# Autodesk Inventor assembly: RobotMK2
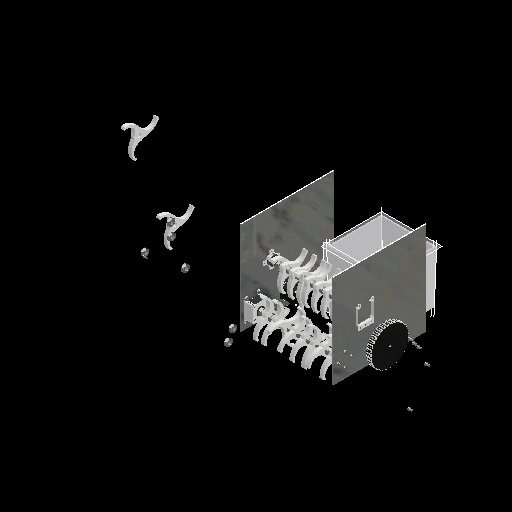
[picture p0: Inventor's stored thumbnail of the model, 512x512]
Saved by Autodesk Inventor 2025 (Build 290162000, 162)
## iProperties
Created: 2025-01-19
Part Number: RobotMK2
Document SubType Name: Assembly
Designer: Trevor
Author: Trevor
## Documents named in this file (18)
- C:\Users\Trevor\Documents\GitHub\USA-Robotic-Club-2024\assests\RobotMK2.iam
- C:\Users\Trevor\Documents\GitHub\USA-Robotic-Club-2024\assests\RightALPanel.ipt
- C:\Users\Trevor\Documents\GitHub\USA-Robotic-Club-2024\assests\LeftALPanel.ipt
- C:\Users\Trevor\Documents\GitHub\USA-Robotic-Club-2024\assests\RobotWheelMK1.ipt
- C:\Users\Trevor\Documents\GitHub\USA-Robotic-Club-2024\assests\Robot Box.ipt
- C:\Users\Trevor\Documents\GitHub\USA-Robotic-Club-2024\assests\17hm08-1204s-nema17-pancake-21mm-1.snapshot.2\17HM08-1204S Nema17 Pancake 21mm\17HM08-1204S Nema17 Pancake 21mm.ipt
- C:\Users\Trevor\Documents\GitHub\USA-Robotic-Club-2024\assests\stepperonline-nema-17-1.snapshot.1\Stepper Motor\Stepper Motor.ipt
- C:\Users\Trevor\Documents\GitHub\USA-Robotic-Club-2024\assests\RodMK3.ipt
- C:\Users\Trevor\Documents\GitHub\USA-Robotic-Club-2024\assests\Combine mk5.ipt
- C:\Users\Trevor\Documents\GitHub\USA-Robotic-Club-2024\assests\bearing-10mm-2.snapshot.2\PMG(Si)\PMG(Si).ipt
- C:\Users\Trevor\Documents\Inventor\Content Center Files\R2025\en-US\DIN 934\DIN 934 - M10 x 1.ipt
- C:\Users\Trevor\Documents\GitHub\USA-Robotic-Club-2024\assests\PanpackeMotorMountMK2.ipt
- C:\Users\Trevor\Documents\GitHub\USA-Robotic-Club-2024\assests\BearingMountMK2.ipt
- C:\Users\Trevor\Documents\Inventor\Content Center Files\R2025\en-US\ANSI B18.3.4M(1)\ANSI B18.3.4M - M5 x 0.8 x 8(2).ipt
- C:\Users\Trevor\Documents\Inventor\Content Center Files\R2025\en-US\DIN 934\DIN 934 - M5 x 0.8.ipt
- C:\Users\Trevor\Documents\Inventor\Content Center Files\R2025\en-US\ANSI B18.3.4M(1)\ANSI B18.3.4M - M3 x 0.5 x 10(2).ipt
- C:\Users\Trevor\Documents\Inventor\Content Center Files\R2025\en-US\ANSI B18.3.4M(1)\ANSI B18.3.4M - M5 x 0.8 x 10(2).ipt
- C:\Users\Trevor\Documents\GitHub\USA-Robotic-Club-2024\assests\Bucket no fillets 2.ipt
## Components (108 placed, 17 different names)
1. Robot Box:1 — Mate:1, Mate:2, Mate:3, Mate:4, Mate:5, Mate:6, Mate:7, Flush:3, Flush:4, Mate:12
2. RobotWheelMK1:1 — Mate:2, Mate:3, Mate:4, Flush:1, Mate:8
3. RobotWheelMK1:2 — Mate:5, Mate:6, Mate:7, Mate:10
4. RightALPanel:1 — Flush:5, Mate:9, Mate:21, Flush:11, Mate:74, Mate:76, Mate:77, Mate:79, Mate:81, Mate:82, Mate:83, Mate:88, Mate:91, Mate:92, Mate:93, Mate:94, Mate:95, Mate:96, Mate:97, Mate:131
5. LeftALPanel:1 — Flush:6, Mate:11, Mate:17, Flush:7, Flush:10, Mate:98, Mate:99, Mate:100, Mate:101, Mate:102, Mate:103, Mate:104, Mate:105, Mate:106, Mate:107, Mate:108, Mate:116, Mate:117, Mate:118, Mate:122, Mate:124, Mate:127, Mate:128, Mate:129, Mate:132, Mate:133
6. Stepper Motor:1 — Mate:8, Mate:9, Mate:13, Mate:90
7. Stepper Motor:2 — Mate:10, Mate:11, Mate:12, Mate:13
8. RodMK3:1 — Mate:18, Mate:19, Mate:20, Mate:24, Mate:26, Mate:28, Mate:29, Mate:30, Mate:31, Mate:33, Mate:34, Mate:38, Mate:39, Mate:43, Mate:44, Mate:48, Mate:50, Mate:52, Mate:54, Mate:55, Mate:58, Mate:60, Mate:61, Mate:64, Mate:66, Mate:67, Mate:70, Mate:72
9. 17HM08-1204S Nema17 Pancake 21mm:1 — Mate:17, Mate:18, Mate:19, Flush:8, Flush:9
10. PMG(Si):1 — Mate:20, Mate:21
11. DIN 934 - replaced by DIN EN 24032/28673/28674 M10 x 1:1 — Mate:24, Mate:27
12. DIN 934 - replaced by DIN EN 24032/28673/28674 M10 x 1:2 — Mate:26, Mate:27, Mate:32
13. DIN 934 - replaced by DIN EN 24032/28673/28674 M10 x 1:4 — Mate:48, Mate:49, Mate:51
14. DIN 934 - replaced by DIN EN 24032/28673/28674 M10 x 1:3 — Mate:33, Mate:35, Mate:36
15. DIN 934 - replaced by DIN EN 24032/28673/28674 M10 x 1:5 — Mate:34, Mate:36, Mate:37
16. DIN 934 - replaced by DIN EN 24032/28673/28674 M10 x 1:6 — Mate:38, Mate:40, Mate:41
17. DIN 934 - replaced by DIN EN 24032/28673/28674 M10 x 1:7 — Mate:50, Mate:51, Mate:53
18. DIN 934 - replaced by DIN EN 24032/28673/28674 M10 x 1:8 — Mate:44, Mate:46, Mate:47
19. DIN 934 - replaced by DIN EN 24032/28673/28674 M10 x 1:9 — Mate:43, Mate:45, Mate:46
20. DIN 934 - replaced by DIN EN 24032/28673/28674 M10 x 1:10 — Mate:39, Mate:41, Mate:42
21. DIN 934 - replaced by DIN EN 24032/28673/28674 M10 x 1:11 — Mate:60, Mate:62, Mate:63
22. DIN 934 - replaced by DIN EN 24032/28673/28674 M10 x 1:12 — Mate:66, Mate:68, Mate:69
23. Combine mk5:2 — Mate:28, Mate:32, Mate:35
24. Combine mk5:3 — Mate:29, Mate:37, Mate:40
25. Combine mk5:4 — Mate:30, Mate:42, Mate:45
26. Combine mk5:5 — Mate:31, Mate:47, Mate:49
27. Combine mk5:6 — Mate:146, Mate:147, Mate:149
28. Combine mk5:7 — Mate:70, Mate:71, Mate:73
29. Combine mk5:8 — Mate:58, Mate:59, Mate:62
30. Combine mk5:9 — Mate:64, Mate:65, Mate:68
31. Combine mk5:10 — Mate:140, Mate:141, Mate:143
32. Combine mk5:11 — Mate:52, Mate:53, Mate:56
33. DIN 934 - replaced by DIN EN 24032/28673/28674 M10 x 1:13 — Mate:61, Mate:63, Mate:65
34. DIN 934 - replaced by DIN EN 24032/28673/28674 M10 x 1:14 — Mate:67, Mate:69, Mate:71
35. DIN 934 - replaced by DIN EN 24032/28673/28674 M10 x 1:15 — Mate:160, Mate:161, Mate:163
36. DIN 934 - replaced by DIN EN 24032/28673/28674 M10 x 1:16 — Mate:144, Mate:145, Mate:147
37. DIN 934 - replaced by DIN EN 24032/28673/28674 M10 x 1:17 — Mate:54, Mate:56, Mate:57
38. DIN 934 - replaced by DIN EN 24032/28673/28674 M10 x 1:18 — Mate:55, Mate:57, Mate:59
39. DIN 934 - replaced by DIN EN 24032/28673/28674 M10 x 1:19 — Mate:72, Mate:73
40. DIN 934 - replaced by DIN EN 24032/28673/28674 M10 x 1:20 — Mate:138, Mate:139, Mate:141
41. DIN 934 - replaced by DIN EN 24032/28673/28674 M10 x 1:21 — Mate:142, Mate:143, Mate:145
42. PanpackeMotorMountMK2:1 — Flush:9, Flush:10, Mate:109, Mate:110, Mate:111, Mate:112, Mate:113, Mate:114, Mate:115
43. BearingMountMK2:1 — Flush:11, Mate:75, Mate:78, Mate:80, Mate:126
44. Broached Hexagon Socket Button Head Cap Screw - Metric M5 x 0.8 x 10:8 — Mate:74, Mate:75, Mate:84
45. Broached Hexagon Socket Button Head Cap Screw - Metric M5 x 0.8 x 10:9 — Mate:76, Mate:85, Mate:126
46. Broached Hexagon Socket Button Head Cap Screw - Metric M5 x 0.8 x 8:3
47. Broached Hexagon Socket Button Head Cap Screw - Metric M5 x 0.8 x 10:1 — Mate:106, Mate:115, Mate:125
48. Broached Hexagon Socket Button Head Cap Screw - Metric M5 x 0.8 x 10:7 — Mate:77, Mate:78, Mate:89
49. Broached Hexagon Socket Button Head Cap Screw - Metric M5 x 0.8 x 8:6
50. Broached Hexagon Socket Button Head Cap Screw - Metric M5 x 0.8 x 8:7
51. Broached Hexagon Socket Button Head Cap Screw - Metric M5 x 0.8 x 10:6 — Mate:79, Mate:80, Mate:87
52. Broached Hexagon Socket Button Head Cap Screw - Metric M5 x 0.8 x 8:9
53. Broached Hexagon Socket Button Head Cap Screw - Metric M5 x 0.8 x 8:10
54. DIN 934 - replaced by DIN EN 24032/28673/28674 M5:1 — Mate:82, Mate:85
55. DIN 934 - replaced by DIN EN 24032/28673/28674 M5:2 — Mate:81, Mate:84
56. DIN 934 - replaced by DIN EN 24032/28673/28674 M5:4 — Mate:83, Mate:87
57. DIN 934 - replaced by DIN EN 24032/28673/28674 M5:5 — Mate:88, Mate:89
58. Broached Hexagon Socket Button Head Cap Screw - Metric M3 x 0.5 x 10:1 — Mate:94, Mate:96
59. Broached Hexagon Socket Button Head Cap Screw - Metric M3 x 0.5 x 10:2 — Mate:93, Mate:95
60. Broached Hexagon Socket Button Head Cap Screw - Metric M3 x 0.5 x 10:3
61. Broached Hexagon Socket Button Head Cap Screw - Metric M3 x 0.5 x 10:4 — Mate:92, Mate:97
62. Broached Hexagon Socket Button Head Cap Screw - Metric M3 x 0.5 x 10:5 — Mate:90, Mate:91
63. Broached Hexagon Socket Button Head Cap Screw - Metric M3 x 0.5 x 10:7 — Mate:98, Mate:102
64. Broached Hexagon Socket Button Head Cap Screw - Metric M3 x 0.5 x 10:8 — Mate:99, Mate:104
65. Broached Hexagon Socket Button Head Cap Screw - Metric M3 x 0.5 x 10:9 — Mate:100, Mate:105
66. Broached Hexagon Socket Button Head Cap Screw - Metric M3 x 0.5 x 10:10 — Mate:101, Mate:103
67. Broached Hexagon Socket Button Head Cap Screw - Metric M5 x 0.8 x 10:2 — Mate:107, Mate:114, Mate:121
68. Broached Hexagon Socket Button Head Cap Screw - Metric M5 x 0.8 x 10:3 — Mate:108, Mate:113, Mate:123
69. Broached Hexagon Socket Button Head Cap Screw - Metric M5 x 0.8 x 10:4 — Mate:109, Mate:112, Mate:119
70. Broached Hexagon Socket Button Head Cap Screw - Metric M5 x 0.8 x 10:5 — Mate:110, Mate:111, Mate:120
71. DIN 934 - replaced by DIN EN 24032/28673/28674 M5:6 — Mate:118, Mate:121
72. DIN 934 - replaced by DIN EN 24032/28673/28674 M5:7 — Mate:117, Mate:119
73. DIN 934 - replaced by DIN EN 24032/28673/28674 M5:8 — Mate:122, Mate:123
74. DIN 934 - replaced by DIN EN 24032/28673/28674 M5:10 — Mate:116, Mate:120
75. DIN 934 - replaced by DIN EN 24032/28673/28674 M5:11 — Mate:124, Mate:125
76. PanpackeMotorMountMK2:2 — Mate:136, Mate:137
77. PMG(Si):2 — Mate:127, Mate:128, Mate:130
78. BearingMountMK2:2 — Mate:129, Mate:130
79. RodMK3:2 — Mate:133, Mate:134, Mate:135, Mate:138, Mate:140, Mate:142, Mate:144, Mate:146, Mate:148, Mate:150, Mate:152, Mate:154, Mate:155, Mate:157, Mate:160, Mate:162, Mate:164, Mate:166, Mate:168, Mate:170, Mate:171, Mate:172, Mate:175, Mate:177, Mate:178, Mate:181, Mate:183, Mate:184
80. 17HM08-1204S Nema17 Pancake 21mm:2 — Mate:131, Mate:132, Mate:134, Mate:135, Mate:136, Mate:137, Mate:139
81. DIN 934 - replaced by DIN EN 24032/28673/28674 M10 x 1:22 — Mate:148, Mate:149, Mate:151
82. DIN 934 - replaced by DIN EN 24032/28673/28674 M10 x 1:23 — Mate:150, Mate:151, Mate:153
83. DIN 934 - replaced by DIN EN 24032/28673/28674 M10 x 1:24 — Mate:155, Mate:156, Mate:158
84. DIN 934 - replaced by DIN EN 24032/28673/28674 M10 x 1:25 — Mate:157, Mate:158, Mate:159
85. DIN 934 - replaced by DIN EN 24032/28673/28674 M10 x 1:26 — Mate:162, Mate:163, Mate:165
86. DIN 934 - replaced by DIN EN 24032/28673/28674 M10 x 1:27
87. Combine mk5:12 — Mate:152, Mate:153, Mate:156
88. Combine mk5:13 — Mate:154, Mate:159, Mate:161
89. Combine mk5:14 — Mate:164, Mate:165, Mate:167
90. Combine mk5:15 — Mate:170, Mate:173
91. Combine mk5:16
92. Combine mk5:17 — Mate:181, Mate:182, Mate:185
93. Combine mk5:19 — Mate:175, Mate:176, Mate:179
94. Combine mk5:20
95. DIN 934 - replaced by DIN EN 24032/28673/28674 M10 x 1:28
96. DIN 934 - replaced by DIN EN 24032/28673/28674 M10 x 1:29 — Mate:168, Mate:169
97. DIN 934 - replaced by DIN EN 24032/28673/28674 M10 x 1:30 — Mate:178, Mate:179, Mate:180
98. DIN 934 - replaced by DIN EN 24032/28673/28674 M10 x 1:31 — Mate:172, Mate:174, Mate:176
99. DIN 934 - replaced by DIN EN 24032/28673/28674 M10 x 1:32
100. DIN 934 - replaced by DIN EN 24032/28673/28674 M10 x 1:33 — Mate:184, Mate:186
101. DIN 934 - replaced by DIN EN 24032/28673/28674 M10 x 1:34
102. DIN 934 - replaced by DIN EN 24032/28673/28674 M10 x 1:36 — Mate:171, Mate:173, Mate:174
103. DIN 934 - replaced by DIN EN 24032/28673/28674 M10 x 1:37 — Mate:183, Mate:185, Mate:186
104. DIN 934 - replaced by DIN EN 24032/28673/28674 M10 x 1:38 — Mate:166, Mate:167, Mate:169
105. DIN 934 - replaced by DIN EN 24032/28673/28674 M10 x 1:39
106. DIN 934 - replaced by DIN EN 24032/28673/28674 M10 x 1:40
107. DIN 934 - replaced by DIN EN 24032/28673/28674 M10 x 1:41 — Mate:177, Mate:180, Mate:182
108. Bucket no fillets 2:1
## Relationships (189: Mate 179, Flush 10)
- Mate:1: Robot Box:1
- Mate:2: Robot Box:1 ↔ RobotWheelMK1:1
- Mate:3 (2 mm): Robot Box:1 ↔ RobotWheelMK1:1
- Mate:4: Robot Box:1 ↔ RobotWheelMK1:1
- Mate:5: Robot Box:1 ↔ RobotWheelMK1:2
- Mate:6 (2 mm): Robot Box:1 ↔ RobotWheelMK1:2
- Mate:7: Robot Box:1 ↔ RobotWheelMK1:2
- Flush:1 (2 mm): RobotWheelMK1:1
- Flush:3 (20 mm): Robot Box:1
- Flush:4 (30 mm): Robot Box:1
- Flush:5: RightALPanel:1
- Flush:6: LeftALPanel:1
- Mate:8: RobotWheelMK1:1 ↔ Stepper Motor:1
- Mate:9: RightALPanel:1 ↔ Stepper Motor:1
- Mate:10: RobotWheelMK1:2 ↔ Stepper Motor:2
- Mate:11: LeftALPanel:1 ↔ Stepper Motor:2
- Mate:12: Robot Box:1 ↔ Stepper Motor:2
- Mate:13: Stepper Motor:1 ↔ Stepper Motor:2
- Mate:17: LeftALPanel:1 ↔ 17HM08-1204S Nema17 Pancake 21mm:1
- Mate:18: RodMK3:1 ↔ 17HM08-1204S Nema17 Pancake 21mm:1
- Mate:19: RodMK3:1 ↔ 17HM08-1204S Nema17 Pancake 21mm:1
- Flush:7 (-10 mm): LeftALPanel:1
- Flush:8: 17HM08-1204S Nema17 Pancake 21mm:1
- Mate:20: RodMK3:1 ↔ PMG(Si):1
- Mate:21: RightALPanel:1 ↔ PMG(Si):1
- Mate:24: RodMK3:1 ↔ DIN 934 - replaced by DIN EN 24032/28673/28674 M10 x 1:1
- Mate:26: RodMK3:1 ↔ DIN 934 - replaced by DIN EN 24032/28673/28674 M10 x 1:2
- Mate:27: DIN 934 - replaced by DIN EN 24032/28673/28674 M10 x 1:1 ↔ DIN 934 - replaced by DIN EN 24032/28673/28674 M10 x 1:2
- Mate:28: RodMK3:1 ↔ Combine mk5:2
- Mate:29: RodMK3:1 ↔ Combine mk5:3
- Mate:30: RodMK3:1 ↔ Combine mk5:4
- Mate:31: RodMK3:1 ↔ Combine mk5:5
- Mate:32: DIN 934 - replaced by DIN EN 24032/28673/28674 M10 x 1:2 ↔ Combine mk5:2
- Mate:33: RodMK3:1 ↔ DIN 934 - replaced by DIN EN 24032/28673/28674 M10 x 1:3
- Mate:34: RodMK3:1 ↔ DIN 934 - replaced by DIN EN 24032/28673/28674 M10 x 1:5
- Mate:35: DIN 934 - replaced by DIN EN 24032/28673/28674 M10 x 1:3 ↔ Combine mk5:2
- Mate:36: DIN 934 - replaced by DIN EN 24032/28673/28674 M10 x 1:3 ↔ DIN 934 - replaced by DIN EN 24032/28673/28674 M10 x 1:5
- Mate:37: DIN 934 - replaced by DIN EN 24032/28673/28674 M10 x 1:5 ↔ Combine mk5:3
- Mate:38: RodMK3:1 ↔ DIN 934 - replaced by DIN EN 24032/28673/28674 M10 x 1:6
- Mate:39: RodMK3:1 ↔ DIN 934 - replaced by DIN EN 24032/28673/28674 M10 x 1:10
- Mate:40: DIN 934 - replaced by DIN EN 24032/28673/28674 M10 x 1:6 ↔ Combine mk5:3
- Mate:41: DIN 934 - replaced by DIN EN 24032/28673/28674 M10 x 1:6 ↔ DIN 934 - replaced by DIN EN 24032/28673/28674 M10 x 1:10
- Mate:42: DIN 934 - replaced by DIN EN 24032/28673/28674 M10 x 1:10 ↔ Combine mk5:4
- Mate:43: RodMK3:1 ↔ DIN 934 - replaced by DIN EN 24032/28673/28674 M10 x 1:9
- Mate:44: RodMK3:1 ↔ DIN 934 - replaced by DIN EN 24032/28673/28674 M10 x 1:8
- Mate:45: DIN 934 - replaced by DIN EN 24032/28673/28674 M10 x 1:9 ↔ Combine mk5:4
- Mate:46: DIN 934 - replaced by DIN EN 24032/28673/28674 M10 x 1:8 ↔ DIN 934 - replaced by DIN EN 24032/28673/28674 M10 x 1:9
- Mate:47: DIN 934 - replaced by DIN EN 24032/28673/28674 M10 x 1:8 ↔ Combine mk5:5
- Mate:48: RodMK3:1 ↔ DIN 934 - replaced by DIN EN 24032/28673/28674 M10 x 1:4
- Mate:49: DIN 934 - replaced by DIN EN 24032/28673/28674 M10 x 1:4 ↔ Combine mk5:5
- Mate:50: RodMK3:1 ↔ DIN 934 - replaced by DIN EN 24032/28673/28674 M10 x 1:7
- Mate:51: DIN 934 - replaced by DIN EN 24032/28673/28674 M10 x 1:4 ↔ DIN 934 - replaced by DIN EN 24032/28673/28674 M10 x 1:7
- Mate:52: RodMK3:1 ↔ Combine mk5:11
- Mate:53: DIN 934 - replaced by DIN EN 24032/28673/28674 M10 x 1:7 ↔ Combine mk5:11
- Mate:54: RodMK3:1 ↔ DIN 934 - replaced by DIN EN 24032/28673/28674 M10 x 1:17
- Mate:55: RodMK3:1 ↔ DIN 934 - replaced by DIN EN 24032/28673/28674 M10 x 1:18
- Mate:56: Combine mk5:11 ↔ DIN 934 - replaced by DIN EN 24032/28673/28674 M10 x 1:17
- Mate:57: DIN 934 - replaced by DIN EN 24032/28673/28674 M10 x 1:17 ↔ DIN 934 - replaced by DIN EN 24032/28673/28674 M10 x 1:18
- Mate:58: RodMK3:1 ↔ Combine mk5:8
- Mate:59: Combine mk5:8 ↔ DIN 934 - replaced by DIN EN 24032/28673/28674 M10 x 1:18
- Mate:60: RodMK3:1 ↔ DIN 934 - replaced by DIN EN 24032/28673/28674 M10 x 1:11
- Mate:61: RodMK3:1 ↔ DIN 934 - replaced by DIN EN 24032/28673/28674 M10 x 1:13
- Mate:62: DIN 934 - replaced by DIN EN 24032/28673/28674 M10 x 1:11 ↔ Combine mk5:8
- Mate:63: DIN 934 - replaced by DIN EN 24032/28673/28674 M10 x 1:11 ↔ DIN 934 - replaced by DIN EN 24032/28673/28674 M10 x 1:13
- Mate:64: RodMK3:1 ↔ Combine mk5:9
- Mate:65: Combine mk5:9 ↔ DIN 934 - replaced by DIN EN 24032/28673/28674 M10 x 1:13
- Mate:66: RodMK3:1 ↔ DIN 934 - replaced by DIN EN 24032/28673/28674 M10 x 1:12
- Mate:67: RodMK3:1 ↔ DIN 934 - replaced by DIN EN 24032/28673/28674 M10 x 1:14
- Mate:68: DIN 934 - replaced by DIN EN 24032/28673/28674 M10 x 1:12 ↔ Combine mk5:9
- Mate:69: DIN 934 - replaced by DIN EN 24032/28673/28674 M10 x 1:12 ↔ DIN 934 - replaced by DIN EN 24032/28673/28674 M10 x 1:14
- Mate:70: RodMK3:1 ↔ Combine mk5:7
- Mate:71: Combine mk5:7 ↔ DIN 934 - replaced by DIN EN 24032/28673/28674 M10 x 1:14
- Mate:72: RodMK3:1 ↔ DIN 934 - replaced by DIN EN 24032/28673/28674 M10 x 1:19
- Mate:73: Combine mk5:7 ↔ DIN 934 - replaced by DIN EN 24032/28673/28674 M10 x 1:19
- Flush:9: 17HM08-1204S Nema17 Pancake 21mm:1 ↔ PanpackeMotorMountMK2:1
- Flush:10: LeftALPanel:1 ↔ PanpackeMotorMountMK2:1
- Flush:11: RightALPanel:1 ↔ BearingMountMK2:1
- Mate:74: RightALPanel:1 ↔ Broached Hexagon Socket Button Head Cap Screw - Metric M5 x 0.8 x 10:8
- Mate:75: BearingMountMK2:1 ↔ Broached Hexagon Socket Button Head Cap Screw - Metric M5 x 0.8 x 10:8
- Mate:76: RightALPanel:1 ↔ Broached Hexagon Socket Button Head Cap Screw - Metric M5 x 0.8 x 10:9
- Mate:77: RightALPanel:1 ↔ Broached Hexagon Socket Button Head Cap Screw - Metric M5 x 0.8 x 10:7
- Mate:78: BearingMountMK2:1 ↔ Broached Hexagon Socket Button Head Cap Screw - Metric M5 x 0.8 x 10:7
- Mate:79: RightALPanel:1 ↔ Broached Hexagon Socket Button Head Cap Screw - Metric M5 x 0.8 x 10:6
- Mate:80: BearingMountMK2:1 ↔ Broached Hexagon Socket Button Head Cap Screw - Metric M5 x 0.8 x 10:6
- Mate:81: RightALPanel:1 ↔ DIN 934 - replaced by DIN EN 24032/28673/28674 M5:2
- Mate:82: RightALPanel:1 ↔ DIN 934 - replaced by DIN EN 24032/28673/28674 M5:1
- Mate:83: RightALPanel:1 ↔ DIN 934 - replaced by DIN EN 24032/28673/28674 M5:4
- Mate:84: Broached Hexagon Socket Button Head Cap Screw - Metric M5 x 0.8 x 10:8 ↔ DIN 934 - replaced by DIN EN 24032/28673/28674 M5:2
- Mate:85: Broached Hexagon Socket Button Head Cap Screw - Metric M5 x 0.8 x 10:9 ↔ DIN 934 - replaced by DIN EN 24032/28673/28674 M5:1
- Mate:87: Broached Hexagon Socket Button Head Cap Screw - Metric M5 x 0.8 x 10:6 ↔ DIN 934 - replaced by DIN EN 24032/28673/28674 M5:4
- Mate:88: RightALPanel:1 ↔ DIN 934 - replaced by DIN EN 24032/28673/28674 M5:5
- Mate:89: Broached Hexagon Socket Button Head Cap Screw - Metric M5 x 0.8 x 10:7 ↔ DIN 934 - replaced by DIN EN 24032/28673/28674 M5:5
- Mate:90: Stepper Motor:1 ↔ Broached Hexagon Socket Button Head Cap Screw - Metric M3 x 0.5 x 10:5
- Mate:91: RightALPanel:1 ↔ Broached Hexagon Socket Button Head Cap Screw - Metric M3 x 0.5 x 10:5
- Mate:92: RightALPanel:1 ↔ Broached Hexagon Socket Button Head Cap Screw - Metric M3 x 0.5 x 10:4
- Mate:93: RightALPanel:1 ↔ Broached Hexagon Socket Button Head Cap Screw - Metric M3 x 0.5 x 10:2
- Mate:94: RightALPanel:1 ↔ Broached Hexagon Socket Button Head Cap Screw - Metric M3 x 0.5 x 10:1
- Mate:95: RightALPanel:1 ↔ Broached Hexagon Socket Button Head Cap Screw - Metric M3 x 0.5 x 10:2
- Mate:96: RightALPanel:1 ↔ Broached Hexagon Socket Button Head Cap Screw - Metric M3 x 0.5 x 10:1
- Mate:97: RightALPanel:1 ↔ Broached Hexagon Socket Button Head Cap Screw - Metric M3 x 0.5 x 10:4
- Mate:98: LeftALPanel:1 ↔ Broached Hexagon Socket Button Head Cap Screw - Metric M3 x 0.5 x 10:7
- Mate:99: LeftALPanel:1 ↔ Broached Hexagon Socket Button Head Cap Screw - Metric M3 x 0.5 x 10:8
- Mate:100: LeftALPanel:1 ↔ Broached Hexagon Socket Button Head Cap Screw - Metric M3 x 0.5 x 10:9
- Mate:101: LeftALPanel:1 ↔ Broached Hexagon Socket Button Head Cap Screw - Metric M3 x 0.5 x 10:10
- Mate:102: LeftALPanel:1 ↔ Broached Hexagon Socket Button Head Cap Screw - Metric M3 x 0.5 x 10:7
- Mate:103: LeftALPanel:1 ↔ Broached Hexagon Socket Button Head Cap Screw - Metric M3 x 0.5 x 10:10
- Mate:104: LeftALPanel:1 ↔ Broached Hexagon Socket Button Head Cap Screw - Metric M3 x 0.5 x 10:8
- Mate:105: LeftALPanel:1 ↔ Broached Hexagon Socket Button Head Cap Screw - Metric M3 x 0.5 x 10:9
- Mate:106: LeftALPanel:1 ↔ Broached Hexagon Socket Button Head Cap Screw - Metric M5 x 0.8 x 10:1
- Mate:107: LeftALPanel:1 ↔ Broached Hexagon Socket Button Head Cap Screw - Metric M5 x 0.8 x 10:2
- Mate:108: LeftALPanel:1 ↔ Broached Hexagon Socket Button Head Cap Screw - Metric M5 x 0.8 x 10:3
- Mate:109: PanpackeMotorMountMK2:1 ↔ Broached Hexagon Socket Button Head Cap Screw - Metric M5 x 0.8 x 10:4
- Mate:110: PanpackeMotorMountMK2:1 ↔ Broached Hexagon Socket Button Head Cap Screw - Metric M5 x 0.8 x 10:5
- Mate:111: PanpackeMotorMountMK2:1 ↔ Broached Hexagon Socket Button Head Cap Screw - Metric M5 x 0.8 x 10:5
- Mate:112: PanpackeMotorMountMK2:1 ↔ Broached Hexagon Socket Button Head Cap Screw - Metric M5 x 0.8 x 10:4
- Mate:113: PanpackeMotorMountMK2:1 ↔ Broached Hexagon Socket Button Head Cap Screw - Metric M5 x 0.8 x 10:3
- Mate:114: PanpackeMotorMountMK2:1 ↔ Broached Hexagon Socket Button Head Cap Screw - Metric M5 x 0.8 x 10:2
- Mate:115: PanpackeMotorMountMK2:1 ↔ Broached Hexagon Socket Button Head Cap Screw - Metric M5 x 0.8 x 10:1
- Mate:116: LeftALPanel:1 ↔ DIN 934 - replaced by DIN EN 24032/28673/28674 M5:10
- Mate:117: LeftALPanel:1 ↔ DIN 934 - replaced by DIN EN 24032/28673/28674 M5:7
- Mate:118: LeftALPanel:1 ↔ DIN 934 - replaced by DIN EN 24032/28673/28674 M5:6
- Mate:119: Broached Hexagon Socket Button Head Cap Screw - Metric M5 x 0.8 x 10:4 ↔ DIN 934 - replaced by DIN EN 24032/28673/28674 M5:7
- Mate:120: Broached Hexagon Socket Button Head Cap Screw - Metric M5 x 0.8 x 10:5 ↔ DIN 934 - replaced by DIN EN 24032/28673/28674 M5:10
- Mate:121: Broached Hexagon Socket Button Head Cap Screw - Metric M5 x 0.8 x 10:2 ↔ DIN 934 - replaced by DIN EN 24032/28673/28674 M5:6
- Mate:122: LeftALPanel:1 ↔ DIN 934 - replaced by DIN EN 24032/28673/28674 M5:8
- Mate:123: Broached Hexagon Socket Button Head Cap Screw - Metric M5 x 0.8 x 10:3 ↔ DIN 934 - replaced by DIN EN 24032/28673/28674 M5:8
- Mate:124: LeftALPanel:1 ↔ DIN 934 - replaced by DIN EN 24032/28673/28674 M5:11
- Mate:125: Broached Hexagon Socket Button Head Cap Screw - Metric M5 x 0.8 x 10:1 ↔ DIN 934 - replaced by DIN EN 24032/28673/28674 M5:11
- Mate:126: BearingMountMK2:1 ↔ Broached Hexagon Socket Button Head Cap Screw - Metric M5 x 0.8 x 10:9
- Mate:127: LeftALPanel:1 ↔ PMG(Si):2
- Mate:128: LeftALPanel:1 ↔ PMG(Si):2
- Mate:129: LeftALPanel:1 ↔ BearingMountMK2:2
- Mate:130: PMG(Si):2 ↔ BearingMountMK2:2
- Mate:131: RightALPanel:1 ↔ 17HM08-1204S Nema17 Pancake 21mm:2
- Mate:132: LeftALPanel:1 ↔ 17HM08-1204S Nema17 Pancake 21mm:2
- Mate:133: LeftALPanel:1 ↔ RodMK3:2
- Mate:134: RodMK3:2 ↔ 17HM08-1204S Nema17 Pancake 21mm:2
- Mate:135: RodMK3:2 ↔ 17HM08-1204S Nema17 Pancake 21mm:2
- Mate:136: PanpackeMotorMountMK2:2 ↔ 17HM08-1204S Nema17 Pancake 21mm:2
- Mate:137: PanpackeMotorMountMK2:2 ↔ 17HM08-1204S Nema17 Pancake 21mm:2
- Mate:138: DIN 934 - replaced by DIN EN 24032/28673/28674 M10 x 1:20 ↔ RodMK3:2
- Mate:139: DIN 934 - replaced by DIN EN 24032/28673/28674 M10 x 1:20 ↔ 17HM08-1204S Nema17 Pancake 21mm:2
- Mate:140: Combine mk5:10 ↔ RodMK3:2
- Mate:141: Combine mk5:10 ↔ DIN 934 - replaced by DIN EN 24032/28673/28674 M10 x 1:20
- Mate:142: DIN 934 - replaced by DIN EN 24032/28673/28674 M10 x 1:21 ↔ RodMK3:2
- Mate:143: Combine mk5:10 ↔ DIN 934 - replaced by DIN EN 24032/28673/28674 M10 x 1:21
- Mate:144: DIN 934 - replaced by DIN EN 24032/28673/28674 M10 x 1:16 ↔ RodMK3:2
- Mate:145: DIN 934 - replaced by DIN EN 24032/28673/28674 M10 x 1:16 ↔ DIN 934 - replaced by DIN EN 24032/28673/28674 M10 x 1:21
- Mate:146: Combine mk5:6 ↔ RodMK3:2
- Mate:147: Combine mk5:6 ↔ DIN 934 - replaced by DIN EN 24032/28673/28674 M10 x 1:16
- Mate:148: RodMK3:2 ↔ DIN 934 - replaced by DIN EN 24032/28673/28674 M10 x 1:22
- Mate:149: Combine mk5:6 ↔ DIN 934 - replaced by DIN EN 24032/28673/28674 M10 x 1:22
- Mate:150: RodMK3:2 ↔ DIN 934 - replaced by DIN EN 24032/28673/28674 M10 x 1:23
- Mate:151: DIN 934 - replaced by DIN EN 24032/28673/28674 M10 x 1:22 ↔ DIN 934 - replaced by DIN EN 24032/28673/28674 M10 x 1:23
- Mate:152: RodMK3:2 ↔ Combine mk5:12
- Mate:153: DIN 934 - replaced by DIN EN 24032/28673/28674 M10 x 1:23 ↔ Combine mk5:12
- Mate:154: RodMK3:2 ↔ Combine mk5:13
- Mate:155: RodMK3:2 ↔ DIN 934 - replaced by DIN EN 24032/28673/28674 M10 x 1:24
- Mate:156: DIN 934 - replaced by DIN EN 24032/28673/28674 M10 x 1:24 ↔ Combine mk5:12
- Mate:157: RodMK3:2 ↔ DIN 934 - replaced by DIN EN 24032/28673/28674 M10 x 1:25
- Mate:158: DIN 934 - replaced by DIN EN 24032/28673/28674 M10 x 1:24 ↔ DIN 934 - replaced by DIN EN 24032/28673/28674 M10 x 1:25
- Mate:159: DIN 934 - replaced by DIN EN 24032/28673/28674 M10 x 1:25 ↔ Combine mk5:13
- Mate:160: DIN 934 - replaced by DIN EN 24032/28673/28674 M10 x 1:15 ↔ RodMK3:2
- Mate:161: DIN 934 - replaced by DIN EN 24032/28673/28674 M10 x 1:15 ↔ Combine mk5:13
- Mate:162: RodMK3:2 ↔ DIN 934 - replaced by DIN EN 24032/28673/28674 M10 x 1:26
- Mate:163: DIN 934 - replaced by DIN EN 24032/28673/28674 M10 x 1:15 ↔ DIN 934 - replaced by DIN EN 24032/28673/28674 M10 x 1:26
- Mate:164: RodMK3:2 ↔ Combine mk5:14
- Mate:165: DIN 934 - replaced by DIN EN 24032/28673/28674 M10 x 1:26 ↔ Combine mk5:14
- Mate:166: RodMK3:2 ↔ DIN 934 - replaced by DIN EN 24032/28673/28674 M10 x 1:38
- Mate:167: Combine mk5:14 ↔ DIN 934 - replaced by DIN EN 24032/28673/28674 M10 x 1:38
- Mate:168: RodMK3:2 ↔ DIN 934 - replaced by DIN EN 24032/28673/28674 M10 x 1:29
- Mate:169: DIN 934 - replaced by DIN EN 24032/28673/28674 M10 x 1:29 ↔ DIN 934 - replaced by DIN EN 24032/28673/28674 M10 x 1:38
- Mate:170: RodMK3:2 ↔ Combine mk5:15
- Mate:171: RodMK3:2 ↔ DIN 934 - replaced by DIN EN 24032/28673/28674 M10 x 1:36
- Mate:172: RodMK3:2 ↔ DIN 934 - replaced by DIN EN 24032/28673/28674 M10 x 1:31
- Mate:173: Combine mk5:15 ↔ DIN 934 - replaced by DIN EN 24032/28673/28674 M10 x 1:36
- Mate:174: DIN 934 - replaced by DIN EN 24032/28673/28674 M10 x 1:31 ↔ DIN 934 - replaced by DIN EN 24032/28673/28674 M10 x 1:36
- Mate:175: RodMK3:2 ↔ Combine mk5:19
- Mate:176: Combine mk5:19 ↔ DIN 934 - replaced by DIN EN 24032/28673/28674 M10 x 1:31
- Mate:177: RodMK3:2 ↔ DIN 934 - replaced by DIN EN 24032/28673/28674 M10 x 1:41
- Mate:178: RodMK3:2 ↔ DIN 934 - replaced by DIN EN 24032/28673/28674 M10 x 1:30
- Mate:179: Combine mk5:19 ↔ DIN 934 - replaced by DIN EN 24032/28673/28674 M10 x 1:30
- Mate:180: DIN 934 - replaced by DIN EN 24032/28673/28674 M10 x 1:30 ↔ DIN 934 - replaced by DIN EN 24032/28673/28674 M10 x 1:41
- Mate:181: RodMK3:2 ↔ Combine mk5:17
- Mate:182: Combine mk5:17 ↔ DIN 934 - replaced by DIN EN 24032/28673/28674 M10 x 1:41
- Mate:183: RodMK3:2 ↔ DIN 934 - replaced by DIN EN 24032/28673/28674 M10 x 1:37
- Mate:184: RodMK3:2 ↔ DIN 934 - replaced by DIN EN 24032/28673/28674 M10 x 1:33
- Mate:185: Combine mk5:17 ↔ DIN 934 - replaced by DIN EN 24032/28673/28674 M10 x 1:37
- Mate:186: DIN 934 - replaced by DIN EN 24032/28673/28674 M10 x 1:33 ↔ DIN 934 - replaced by DIN EN 24032/28673/28674 M10 x 1:37
